# Autodesk Inventor assembly: XY Joint Left
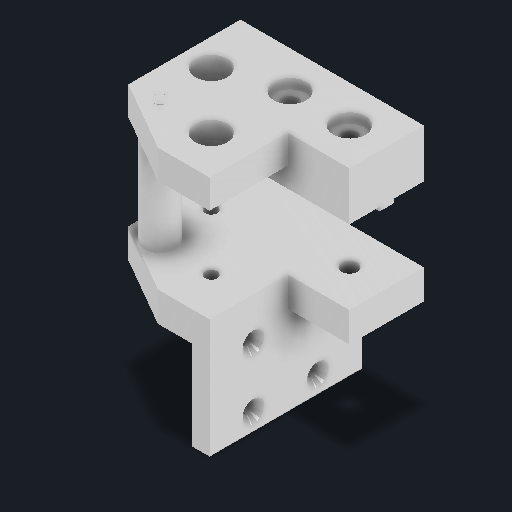
[picture p0: Inventor's stored thumbnail of the model, 512x512]
Saved by Autodesk Inventor 2025.1 (Build 291241020, 241B)
## iProperties
Created: 2025-04-19
Part Number: XY Joint Left
Document SubType Name: Assembly
Designer: Joshua Eah
Author: Joshua Eah
## Documents named in this file (5)
- C:\Users\Joshua Eah\Documents\Voron 0.2\CAD\Machined Parts\XY Joints\XY Joint Left\XY Joint Left.iam
- XY Joint Left.iam
- C:\Users\Joshua Eah\Documents\Voron 0.2\CAD\Machined Parts\XY Joints\XY Joint Left\XY Joint Left Lower.ipt
- C:\Users\Joshua Eah\Documents\Voron 0.2\CAD\Machined Parts\XY Joints\XY Joint Left\XY Joint Left Upper.ipt
- C:\Users\Joshua Eah\Documents\Voron 0.2\CAD\Machined Parts\XY Joints\XY Joint Support\XY Joint Support.ipt
## Components (3 placed, 3 different names)
1. XY Joint Left Lower:1 — Rotational:1
2. XY Joint Left Upper:1 — Rotational:2
3. XY Joint Support:1 — Rotational:1, Rotational:2
## Relationships (2: RevoluteJoint 2)
- Rotational:1 [RevoluteJoint]: XY Joint Left Lower:1 ↔ XY Joint Support:1
- Rotational:2 [RevoluteJoint]: XY Joint Left Upper:1 ↔ XY Joint Support:1
